# Autodesk Inventor assembly: Dribbler
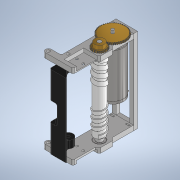
[picture p0: Inventor's stored thumbnail of the model, 180x180]
Saved by Autodesk Inventor 2020.2 (Build 242310000, 310)
## iProperties
Created: 2020-12-03
Part Number: Dribbler
Document SubType Name: Assembly
Designer: Acer
Author: Acer
## Documents named in this file (11)
- C:\Users\Acer\Desktop\2020 LARC\2020_LARC\first_floor\Dribbler\Dribbler.iam
- C:\Users\Acer\Desktop\2020 LARC\2020_LARC\first_floor\Dribbler\PartA.ipt
- C:\Users\Acer\Desktop\2020 LARC\2020_LARC\first_floor\Dribbler\PartB.ipt
- C:\Users\Acer\Desktop\2020 LARC\2020_LARC\first_floor\Dribbler\PartC.ipt
- C:\Users\Acer\Desktop\2020 LARC\2020_LARC\first_floor\Dribbler\Kugellager 685-ZZ-C3.ipt
- C:\Users\Acer\Desktop\2020 LARC\2020_LARC\first_floor\Dribbler\MaxonECmax22-25W.ipt
- C:\Users\Acer\Desktop\2020 LARC\2020_LARC\first_floor\Dribbler\Eixo.ipt
- C:\Users\Acer\Desktop\2020 LARC\2020_LARC\first_floor\Dribbler\Ritzel schmal z26_machined.ipt
- C:\Users\Acer\Desktop\2020 LARC\2020_LARC\first_floor\Dribbler\Ritzel schmal z50.ipt
- C:\Users\Acer\Desktop\2020 LARC\2020_LARC\first_floor\Dribbler\Dribblerschnecke.ipt
- C:\Users\Acer\Desktop\2020 LARC\2020_LARC\first_floor\Dribbler\ChipKicker_v2020_3D.ipt
## Components (11 placed, 10 different names)
1. PartA:1 — Mate:1, Mate:2, Mate:3, Mate:5, Mate:6, Flush:2, Mate:8, Mate:9, Mate:10, Mate:15, Mate:17, Mate:19, Mate:20
2. PartB:1 — Mate:1, Mate:7, Flush:1, Mate:18
3. PartC:1 — Mate:2, Mate:3, Mate:5, Mate:18, Angle:1
4. Kugellager 685-ZZ-C3:1 — Mate:7, Flush:1
5. Kugellager 685-ZZ-C3:2 — Mate:6, Flush:2, Mate:11, Mate:12
6. MaxonECmax22-25W:1 — Mate:8, Mate:9, Mate:10, Mate:14
7. Eixo:1 — Mate:11, Mate:12, Mate:13, Flush:3, Mate:16, Rotation:1, Rotation:2
8. Ritzel schmal z=26:1 — Mate:13, Flush:3, Rotation:2, Rotation:3
9. Ritzel schmal z=50:1 — Mate:14, Mate:15, Rotation:3
10. Dribblerschnecke:1 — Mate:16, Mate:17, Rotation:1
11. ChipKicker_v2020_3D:1 — Mate:19, Mate:20, Angle:1
## Relationships (26: Mate 19, Flush 3, RelateRotation 3, Angle 1)
- Mate:1: PartA:1 ↔ PartB:1
- Mate:2: PartA:1 ↔ PartC:1
- Mate:3: PartA:1 ↔ PartC:1
- Mate:5: PartA:1 ↔ PartC:1
- Mate:6: PartA:1 ↔ Kugellager 685-ZZ-C3:2
- Mate:7: PartB:1 ↔ Kugellager 685-ZZ-C3:1
- Flush:1: PartB:1 ↔ Kugellager 685-ZZ-C3:1
- Flush:2: PartA:1 ↔ Kugellager 685-ZZ-C3:2
- Mate:8: PartA:1 ↔ MaxonECmax22-25W:1
- Mate:9: PartA:1 ↔ MaxonECmax22-25W:1
- Mate:10: PartA:1 ↔ MaxonECmax22-25W:1
- Mate:11: Kugellager 685-ZZ-C3:2 ↔ Eixo:1
- Mate:12: Kugellager 685-ZZ-C3:2 ↔ Eixo:1
- Mate:13: Eixo:1 ↔ Ritzel schmal z=26:1
- Flush:3: Eixo:1 ↔ Ritzel schmal z=26:1
- Mate:14: MaxonECmax22-25W:1 ↔ Ritzel schmal z=50:1
- Mate:15: PartA:1 ↔ Ritzel schmal z=50:1
- Mate:16: Eixo:1 ↔ Dribblerschnecke:1
- Mate:17 (0.5 mm): PartA:1 ↔ Dribblerschnecke:1
- Rotation:1 [RelateRotation] (1 ul): Eixo:1 ↔ Dribblerschnecke:1
- Rotation:2 [RelateRotation] (1 ul): Eixo:1 ↔ Ritzel schmal z=26:1
- Rotation:3 [RelateRotation] (1.92 ul): Ritzel schmal z=26:1 ↔ Ritzel schmal z=50:1
- Mate:18: PartB:1 ↔ PartC:1
- Mate:19: PartA:1 ↔ ChipKicker_v2020_3D:1
- Mate:20 (0.5 mm): PartA:1 ↔ ChipKicker_v2020_3D:1
- Angle:1 (0 deg): PartC:1 ↔ ChipKicker_v2020_3D:1
